# Autodesk Inventor assembly: Assembly2
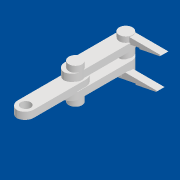
[picture p0: Inventor's stored thumbnail of the model, 180x180]
Saved by Autodesk Inventor 2020 (Build 240168000, 168)
## iProperties
Created: 2022-02-12
Part Number: Assembly2
Document SubType Name: Assembly
Designer: niladri
Author: niladri
## Documents named in this file (4)
- E:\robocon cad model\Assembly2.iam
- E:\robocon cad model\GRIPPER1.ipt
- E:\robocon cad model\GRIPPER3.ipt
- E:\robocon cad model\GRIPPER2.ipt
## Components (7 placed, 3 different names)
1. GRIPPER1:1 — Mate:1
2. GRIPPER1:2
3. GRIPPER1:3
4. GRIPPER3:1 — Mate:1
5. GRIPPER3:2
6. GRIPPER2:2
7. GRIPPER2:3
## Relationships (1: Mate 1)
- Mate:1: GRIPPER1:1 ↔ GRIPPER3:1
